# Autodesk Inventor assembly: Multi-Purpose Custom Bearing Block
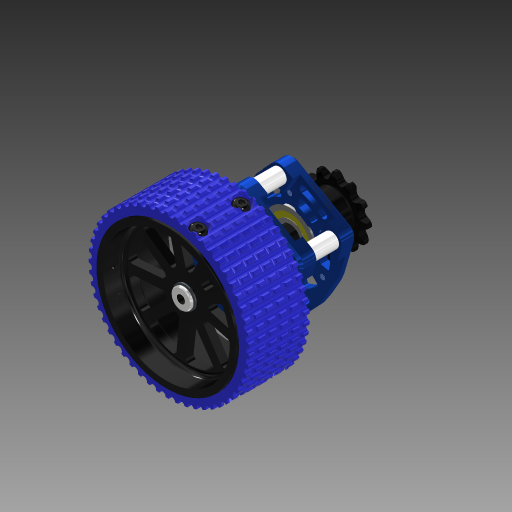
[picture p0: Inventor's stored thumbnail of the model, 512x512]
Saved by Autodesk Inventor 2023 (Build 270158000, 158)
## iProperties
Created: 2022-12-23
Part Number: Multi-Purpose Custom Bearing Block
Document SubType Name: Assembly
Designer: Max Boord
Mass: 533.173 g
Surface Area: 1144.51 cm^2
Volume: 176.819 cm^3
Density: 3.01536 g/cm^3
Author: Max Boord
## iProperties of the stored document MemberDocs/x4kmop1gbL0xjejp40im52g1aKb
Created: 2022-12-23
Part Number: Multi-Purpose Custom Bearing Block
Document SubType Name: Assembly
Designer: Max Boord
Mass: 111.795 g
Surface Area: 267.899 cm^2
Volume: 36.6715 cm^3
Density: 3.04856 g/cm^3
Author: Max Boord
## iProperties of the stored document MemberDocs/x0wjjuorpH0x2k5ka50chthkz3a
Created: 2022-12-23
Part Number: Multi-Purpose Custom Bearing Block
Document SubType Name: Assembly
Designer: Max Boord
Mass: 533.173 g
Surface Area: 1144.51 cm^2
Volume: 176.819 cm^3
Density: 3.01536 g/cm^3
Author: Max Boord
## iProperties of the stored document MemberDocs/xQm4azxvxHk5gsiuaNbdx2mpe5b
Created: 2022-12-23
Part Number: Multi-Purpose Custom Bearing Block
Document SubType Name: Assembly
Designer: Max Boord
Mass: 533.173 g
Surface Area: 1144.51 cm^2
Volume: 176.819 cm^3
Density: 3.01536 g/cm^3
Author: Max Boord
## iProperties of the stored document MemberDocs/xM5epxq2dGk3tsidwUxf1ieijWe
Created: 2022-12-23
Part Number: Multi-Purpose Custom Bearing Block
Document SubType Name: Assembly
Designer: Max Boord
Mass: 533.173 g
Surface Area: 1144.51 cm^2
Volume: 176.819 cm^3
Density: 3.01536 g/cm^3
Author: Max Boord
## Documents named in this file (17)
- E:\Collaborative Robots\Collaborative Part Library\Standard Custom Parts\Plates\Multi-Purpose Custom Bearing Block.iam
- E:\Collaborative Robots\Collaborative Part Library\Standard Custom Parts\Plates\Multi-Purpose Custom Bearing Block.ipt
- E:\Collaborative Robots\Collaborative Part Library\Power Transfer\Bearings and Bushings\Bearings\FR8 (Thunderhex).ipt
- E:\Collaborative Robots\Collaborative Part Library\Power Transfer\Bearings and Bushings\Bearings.ipt
- E:\Collaborative Robots\Collaborative Part Library\Hardware\Fasteners\Machine Screws.ipt
- E:\Collaborative Robots\Collaborative Part Library\Hardware\Spacers\Spacers & Standoffs.ipt
- E:\Collaborative Robots\Collaborative Part Library\Wheels\WCP Nitrile Wheel & Tread.ipt
- E:\Collaborative Robots\Collaborative Part Library\Power Transfer\Sprockets\Sprockets\VexPro 12T 35 Chain 500 Hex Bore Double Sprocket.ipt
- E:\Collaborative Robots\Collaborative Part Library\Power Transfer\Sprockets\VexPro Sprockets.ipt
- E:\Collaborative Robots\Collaborative Part Library\Power Transfer\Hex Spacers.ipt
- E:\Collaborative Robots\Collaborative Part Library\Standard Custom Parts\Plates\Multi-Purpose Custom Bearing Block Shaft.ipt
- E:\Collaborative Robots\Collaborative Part Library\Shaft Retention\Snaprings\Snapring for 0.5in Shaft (0.461in).ipt
- E:\Collaborative Robots\Collaborative Part Library\Shaft Retention\Snaprings.ipt
- E:\Collaborative Robots\Collaborative Part Library\Hardware\Spacers\Spacers & Standoffs\Nylon Unthreaded Spacer (No. 10 x 0.625Lg x 0.375OD).ipt
- E:\Collaborative Robots\Collaborative Part Library\Hardware\Fasteners\Machine Screws\10-32 UNFx1.375 Socket Head Cap Screw.ipt
- E:\Collaborative Robots\Collaborative Part Library\Hardware\Spacers\Spacers & Standoffs\Aluminum Unthreaded Spacer (No. 10 x 1.625Lg x 0.375OD).ipt
- E:\Collaborative Robots\Collaborative Part Library\Hardware\Fasteners\Machine Screws\10-32 UNFx2.5 Socket Head Cap Screw.ipt
## Components (18 placed, 9 different names)
1. Multi-Purpose Custom Bearing Block:1
2. Multi-Purpose Custom Bearing Block:2 — Insert:19
3. FR8 (Thunderhex):1 — Insert:13, Mate:3
4. FR8 (Thunderhex):2 — Insert:12, Insert:19
5. 10-32 UNFx1.375 Socket Head Cap Screw:1
6. 10-32 UNFx1.375 Socket Head Cap Screw:2
7. 10-32 UNFx1.375 Socket Head Cap Screw:3
8. 10-32 UNFx1.375 Socket Head Cap Screw:4
9. Nylon Unthreaded Spacer (No. 10 x 0.625Lg x 0.375OD):1
10. Nylon Unthreaded Spacer (No. 10 x 0.625Lg x 0.375OD):2
11. Nylon Unthreaded Spacer (No. 10 x 0.625Lg x 0.375OD):3
12. Nylon Unthreaded Spacer (No. 10 x 0.625Lg x 0.375OD):4
13. WCP Nitrile Wheel & Tread:1 — Insert:12
14. VexPro 12T 35 Chain 500 Hex Bore Double Sprocket:1 — Insert:20, Insert:21
15. Hex Spacers:1 — Insert:13, Insert:21
16. Multi-Purpose Custom Bearing Block Shaft:1 — Insert:16, Insert:17, Mate:3, Insert:20
17. Snapring for 0.5in Shaft (0.461in):1 — Insert:17
18. Snapring for 0.5in Shaft (0.461in):2 — Insert:16
## Relationships (19: Insert 17, Flush 1, Mate 1)
- [Insert] (25.4 mm): Multi-Purpose Custom Bearing Block:1 ↔ Multi-Purpose Custom Bearing Block:2
- [Flush]: Multi-Purpose Custom Bearing Block:1 ↔ Multi-Purpose Custom Bearing Block:2
- [Insert]: Multi-Purpose Custom Bearing Block:1 ↔ FR8 (Thunderhex):1
- [Insert]: Multi-Purpose Custom Bearing Block:2 ↔ 10-32 UNFx1.375 Socket Head Cap Screw:1
- [Insert]: Multi-Purpose Custom Bearing Block:2 ↔ 10-32 UNFx1.375 Socket Head Cap Screw:4
- [Insert]: Multi-Purpose Custom Bearing Block:2 ↔ 10-32 UNFx1.375 Socket Head Cap Screw:3
- [Insert]: Multi-Purpose Custom Bearing Block:2 ↔ 10-32 UNFx1.375 Socket Head Cap Screw:2
- [Insert]: Multi-Purpose Custom Bearing Block:2 ↔ Nylon Unthreaded Spacer (No. 10 x 0.625Lg x 0.375OD):1
- [Insert]: Multi-Purpose Custom Bearing Block:2 ↔ Nylon Unthreaded Spacer (No. 10 x 0.625Lg x 0.375OD):3
- [Insert]: Multi-Purpose Custom Bearing Block:2 ↔ Nylon Unthreaded Spacer (No. 10 x 0.625Lg x 0.375OD):2
- [Insert]: Multi-Purpose Custom Bearing Block:2 ↔ Nylon Unthreaded Spacer (No. 10 x 0.625Lg x 0.375OD):4
- Insert:12: FR8 (Thunderhex):2 ↔ WCP Nitrile Wheel & Tread:1
- Insert:13: FR8 (Thunderhex):1 ↔ Hex Spacers:1
- Insert:16: Multi-Purpose Custom Bearing Block Shaft:1 ↔ Snapring for 0.5in Shaft (0.461in):2
- Insert:17: Multi-Purpose Custom Bearing Block Shaft:1 ↔ Snapring for 0.5in Shaft (0.461in):1
- Insert:19: Multi-Purpose Custom Bearing Block:2 ↔ FR8 (Thunderhex):2
- Mate:3: FR8 (Thunderhex):1 ↔ Multi-Purpose Custom Bearing Block Shaft:1
- Insert:20: VexPro 12T 35 Chain 500 Hex Bore Double Sprocket:1 ↔ Multi-Purpose Custom Bearing Block Shaft:1
- Insert:21: VexPro 12T 35 Chain 500 Hex Bore Double Sprocket:1 ↔ Hex Spacers:1
## Named parameters: d0_d10 = 0 mm, d1_d11 = 0 mm, d4_d1 = 25.4 mm, d5_d2 = 0 mm
